# Autodesk Inventor assembly: Helping Hand Assembly
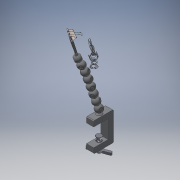
[picture p0: Inventor's stored thumbnail of the model, 180x180]
Saved by Autodesk Inventor 2016 (Build 200138000, 138)
## iProperties
Created: 2017-11-17
Part Number: Helping Hand Assembly
Document SubType Name: Conjunto soldado
Designer: Zigunov
Weld Material: Aço macio soldado
Mass: 43548.6 g
Surface Area: 17698.1 cm^2
Volume: 5533.5 cm^3
Density: 7.87 g/cm^3
Author: Zigunov
## Documents named in this file (7)
- C:\Users\fzigu\Desktop\3D PRINTER\Designs\Lab Items\Helping Hand\Helping Hand Assembly.iam
- C:\Users\fzigu\Desktop\3D PRINTER\Designs\Lab Items\Helping Hand\Table Clamp Strut.ipt
- C:\Users\fzigu\Desktop\3D PRINTER\Designs\Lab Items\Helping Hand\Screw.ipt
- C:\Users\fzigu\Desktop\3D PRINTER\Designs\Lab Items\Helping Hand\Ball Socket.ipt
- C:\Users\fzigu\Desktop\3D PRINTER\Designs\Lab Items\Helping Hand\Table Clamp Swiveling Pad.ipt
- C:\Users\fzigu\Desktop\3D PRINTER\Designs\Lab Items\Helping Hand\Office Clip Receptacle.ipt
- C:\Users\fzigu\Desktop\3D PRINTER\Designs\Lab Items\Helping Hand\Binder Clip.ipt
## Components (12 placed, 6 different names)
1. Table Clamp Strut:1 — Mate:1, Mate:2, Mate:10
2. Screw:1 — Mate:1, Mate:9
3. Ball Socket:1 — Mate:2, Mate:3
4. Ball Socket:2 — Mate:3, Mate:4
5. Ball Socket:3 — Mate:4, Mate:5
6. Ball Socket:4 — Mate:5, Mate:6
7. Ball Socket:5 — Mate:6, Mate:7
8. Ball Socket:6 — Mate:7, Mate:8
9. Ball Socket:7 — Mate:8, Mate:11
10. Table Clamp Swiveling Pad:1 — Mate:9, Mate:10
11. Office Clip Receptacle:1 — Mate:11, Mate:12, Mate:13
12. Binder Clip:1 — Mate:12, Mate:13
## Relationships (13: Mate 13)
- Mate:1: Table Clamp Strut:1 ↔ Screw:1
- Mate:2: Table Clamp Strut:1 ↔ Ball Socket:1
- Mate:3: Ball Socket:1 ↔ Ball Socket:2
- Mate:4: Ball Socket:2 ↔ Ball Socket:3
- Mate:5: Ball Socket:3 ↔ Ball Socket:4
- Mate:6: Ball Socket:4 ↔ Ball Socket:5
- Mate:7: Ball Socket:5 ↔ Ball Socket:6
- Mate:8: Ball Socket:6 ↔ Ball Socket:7
- Mate:9: Screw:1 ↔ Table Clamp Swiveling Pad:1
- Mate:10 (38 mm): Table Clamp Strut:1 ↔ Table Clamp Swiveling Pad:1
- Mate:11: Ball Socket:7 ↔ Office Clip Receptacle:1
- Mate:12: Office Clip Receptacle:1 ↔ Binder Clip:1
- Mate:13: Office Clip Receptacle:1 ↔ Binder Clip:1
